# Autodesk Inventor assembly: EnsamblajeCaja
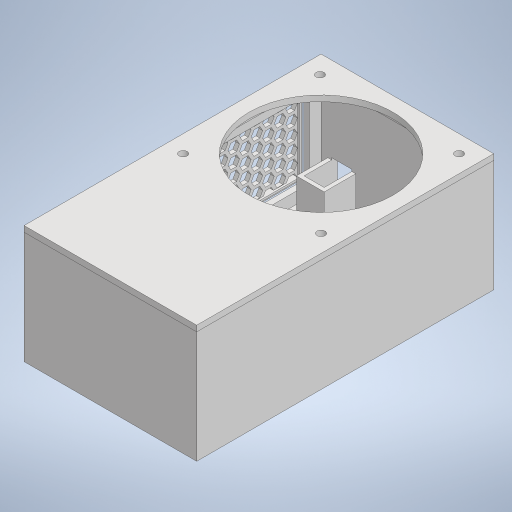
[picture p0: Inventor's stored thumbnail of the model, 512x512]
Saved by Autodesk Inventor 2024 (Build 280153000, 153)
## iProperties
Created: 2023-11-28
Part Number: EnsamblajeCaja
Document SubType Name: Assembly
Designer: sergi
Author: sergi
## Documents named in this file (4)
- C:\Users\sergi\OneDrive\Escritorio\proyectos\3004773_DIY_Dremel_CNC\EnsamblajeCaja.iam
- C:\Users\sergi\OneDrive\Escritorio\proyectos\3004773_DIY_Dremel_CNC\CajaControladora.ipt
- C:\Users\sergi\OneDrive\Escritorio\TapaControladora.ipt
- C:\Users\sergi\OneDrive\Escritorio\Ventilación.ipt
## Components (3 placed, 3 different names)
1. CajaControladora:1 — Nivelación:1, Nivelación:2, Coincidencia:1, Coincidencia:2
2. TapaControladora:1 — Nivelación:1
3. Ventilación:1 — Nivelación:2, Coincidencia:1, Coincidencia:2
## Relationships (4: Flush 2, Mate 2)
- Nivelación:1 [Flush]: CajaControladora:1 ↔ TapaControladora:1
- Nivelación:2 [Flush]: CajaControladora:1 ↔ Ventilación:1
- Coincidencia:1 [Mate] (0.25 mm): CajaControladora:1 ↔ Ventilación:1
- Coincidencia:2 [Mate] (0.25 mm): CajaControladora:1 ↔ Ventilación:1
